# Autodesk Inventor assembly: PCB Component
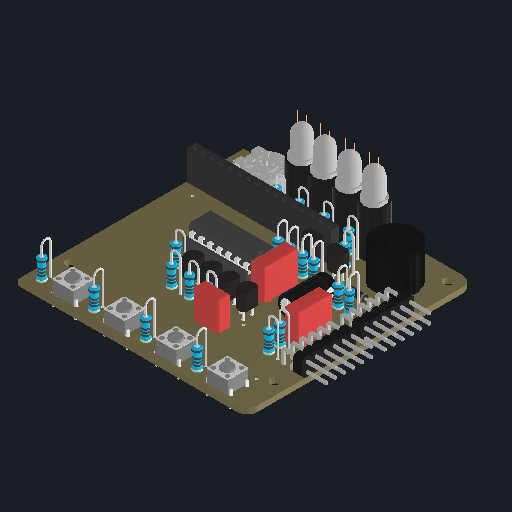
[picture p0: Inventor's stored thumbnail of the model, 512x512]
Saved by Autodesk Inventor 2023 (Build 270158000, 158)
## iProperties
Created: 2022-12-22
Part Number: PCB Component
Document SubType Name: Assembly
Designer: Manuel
Author: Manuel
## Documents named in this file (20)
- C:\workspace\Studium\WST\opcua_netzwerk\Entwicklung Knoten\3D Modell\ConnectorHead_RPi\PCB Component.iam
- C:\workspace\Studium\WST\opcua_netzwerk\Entwicklung Knoten\3D Modell\ConnectorHead_RPi\Board.ipt
- C:\workspace\Studium\WST\opcua_netzwerk\Entwicklung Knoten\3D Modell\ConnectorHead_RPi\2X20.iam
- C:\workspace\Studium\WST\opcua_netzwerk\Entwicklung Knoten\3D Modell\ConnectorHead_RPi\B3F-10XX.iam
- C:\workspace\Studium\WST\opcua_netzwerk\Entwicklung Knoten\3D Modell\ConnectorHead_RPi\1X16F.ipt
- C:\workspace\Studium\WST\opcua_netzwerk\Entwicklung Knoten\3D Modell\ConnectorHead_RPi\F_CM12P.ipt
- C:\workspace\Studium\WST\opcua_netzwerk\Entwicklung Knoten\3D Modell\ConnectorHead_RPi\DIL14.iam
- C:\workspace\Studium\WST\opcua_netzwerk\Entwicklung Knoten\3D Modell\ConnectorHead_RPi\TO92.ipt
- C:\workspace\Studium\WST\opcua_netzwerk\Entwicklung Knoten\3D Modell\ConnectorHead_RPi\PT-10.ipt
- C:\workspace\Studium\WST\opcua_netzwerk\Entwicklung Knoten\3D Modell\ConnectorHead_RPi\DO35-7.ipt
- C:\workspace\Studium\WST\opcua_netzwerk\Entwicklung Knoten\3D Modell\ConnectorHead_RPi\2X06_90.ipt
- C:\workspace\Studium\WST\opcua_netzwerk\Entwicklung Knoten\3D Modell\ConnectorHead_RPi\0309V.ipt
- C:\workspace\Studium\WST\opcua_netzwerk\Entwicklung Knoten\3D Modell\ConnectorHead_RPi\C075-042X103.ipt
- C:\workspace\Studium\WST\opcua_netzwerk\Entwicklung Knoten\3D Modell\ConnectorHead_RPi\C050-035X075.ipt
- C:\workspace\Studium\WST\opcua_netzwerk\Entwicklung Knoten\3D Modell\ConnectorHead_RPi\E2,5-6_FLAT_DOWN.ipt
- C:\workspace\Studium\WST\opcua_netzwerk\Entwicklung Knoten\3D Modell\ConnectorHead_RPi\LEDs\Abstandhalter_13mm.ipt
- C:\workspace\Studium\WST\opcua_netzwerk\Entwicklung Knoten\3D Modell\ConnectorHead_RPi\LEDs\LED - blue.ipt
- C:\workspace\Studium\WST\opcua_netzwerk\Entwicklung Knoten\3D Modell\ConnectorHead_RPi\LEDs\LED - green.ipt
- C:\workspace\Studium\WST\opcua_netzwerk\Entwicklung Knoten\3D Modell\ConnectorHead_RPi\LEDs\LED - red.ipt
- C:\workspace\Studium\WST\opcua_netzwerk\Entwicklung Knoten\3D Modell\ConnectorHead_RPi\LEDs\LED - yellow.ipt
## Components (52 placed, 49 different names)
1. Board:1 — Passend:13, Passend:14, Passend:15, Passend:16, Passend:17, Passend:18, Passend:19, Passend:20, Passend:21
2. 2X20:U$1 [sub-assembly]
3. B3F-10XX:S1 [sub-assembly]
4. B3F-10XX:S2 [sub-assembly]
5. B3F-10XX:S3 [sub-assembly]
6. B3F-10XX:S4 [sub-assembly]
7. 1X16F:JP1
8. F/CM12P:SG1
9. DIL14:IC1 [sub-assembly]
10. TO92:T2
11. TO92:T1
12. TO92:T3
13. TO92:T4
14. TO92:T5
15. TO92:T8
16. PT-10:R9
17. DO35-7:D2
18. 2X06/90:JP2
19. 2X06/90:JP3
20. 0309V:R16
21. 0309V:R14
22. 0309V:R1
23. 0309V:R2
24. 0309V:R3
25. 0309V:R6
26. 0309V:R4
27. 0309V:R5
28. 0309V:R7
29. 0309V:R8
30. 0309V:R15
31. 0309V:R10
32. 0309V:R11
33. 0309V:R12
34. 0309V:R13
35. 0309V:R17
36. 0309V:R18
37. 0309V:R23
38. 0309V:R24
39. 0309V:R19
40. 0309V:R20
41. C075-042X103:C1
42. C075-042X103:C2
43. C050-035X075:C3
44. E2,5-6_FLAT_DOWN:C5
45. Abstandhalter_13mm:1 — Passend:1, Passend:2, Passend:3, Fluchtend:3
46. LED - blue:1 — Passend:1, Passend:2, Passend:3, Passend:13, Passend:14
47. LED - green:1 — Passend:10, Passend:11, Passend:12, Passend:19, Passend:20
48. LED - red:1 — Passend:7, Passend:8, Passend:9, Passend:15, Passend:16
49. LED - yellow:1 — Passend:4, Passend:5, Passend:6, Passend:17, Passend:18
50. Abstandhalter_13mm:2 — Passend:10, Passend:11, Passend:12, Fluchtend:1
51. Abstandhalter_13mm:3 — Passend:7, Passend:8, Passend:9, Fluchtend:2, Fluchtend:3, Passend:21
52. Abstandhalter_13mm:4 — Passend:4, Passend:5, Passend:6, Fluchtend:1, Fluchtend:2
## Relationships (24: Mate 21, Flush 3)
- Passend:1 [Mate]: Abstandhalter_13mm:1 ↔ LED - blue:1
- Passend:2 [Mate]: Abstandhalter_13mm:1 ↔ LED - blue:1
- Passend:3 [Mate]: Abstandhalter_13mm:1 ↔ LED - blue:1
- Passend:4 [Mate]: LED - yellow:1 ↔ Abstandhalter_13mm:4
- Passend:5 [Mate]: LED - yellow:1 ↔ Abstandhalter_13mm:4
- Passend:6 [Mate]: LED - yellow:1 ↔ Abstandhalter_13mm:4
- Passend:7 [Mate]: LED - red:1 ↔ Abstandhalter_13mm:3
- Passend:8 [Mate]: LED - red:1 ↔ Abstandhalter_13mm:3
- Passend:9 [Mate]: LED - red:1 ↔ Abstandhalter_13mm:3
- Passend:10 [Mate]: LED - green:1 ↔ Abstandhalter_13mm:2
- Passend:11 [Mate]: LED - green:1 ↔ Abstandhalter_13mm:2
- Passend:12 [Mate]: LED - green:1 ↔ Abstandhalter_13mm:2
- Passend:13 [Mate]: Board:1 ↔ LED - blue:1
- Passend:14 [Mate]: Board:1 ↔ LED - blue:1
- Passend:15 [Mate]: Board:1 ↔ LED - red:1
- Passend:16 [Mate]: Board:1 ↔ LED - red:1
- Passend:17 [Mate]: Board:1 ↔ LED - yellow:1
- Passend:18 [Mate]: Board:1 ↔ LED - yellow:1
- Passend:19 [Mate]: Board:1 ↔ LED - green:1
- Passend:20 [Mate]: Board:1 ↔ LED - green:1
- Fluchtend:1 [Flush]: Abstandhalter_13mm:2 ↔ Abstandhalter_13mm:4
- Fluchtend:2 [Flush]: Abstandhalter_13mm:3 ↔ Abstandhalter_13mm:4
- Fluchtend:3 [Flush]: Abstandhalter_13mm:1 ↔ Abstandhalter_13mm:3
- Passend:21 [Mate]: Board:1 ↔ Abstandhalter_13mm:3
